# Autodesk Inventor assembly: SimulationWheelAssembly
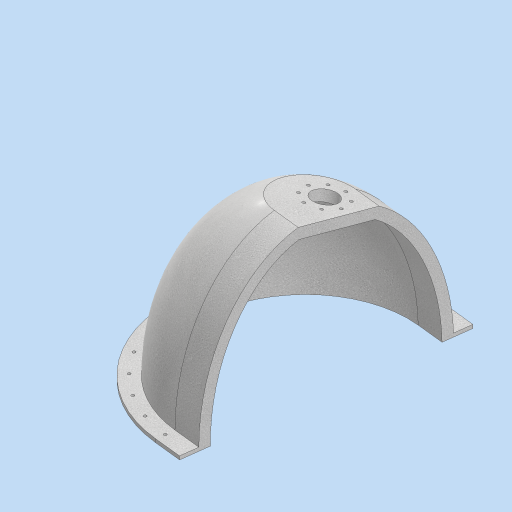
[picture p0: Inventor's stored thumbnail of the model, 512x512]
Saved by Autodesk Inventor 2023 (Build 270158000, 158)
## iProperties
Created: 2026-03-22
Part Number: SimulationWheelAssembly
Document SubType Name: Assembly
Designer: Nathann
Mass: 20175 g
Surface Area: 18221.2 cm^2
Volume: 20175 cm^3
Density: 1 g/cm^3
Author: Nathann
## Documents named in this file (8)
- C:\Users\Nathann\ClawdDrive\Objet3D\neodrive\neodrive-cad-ergonomic-v1\SimulationWheelAssembly.iam
- C:\Users\Nathann\ClawdDrive\Objet3D\neodrive\neodrive-cad-ergonomic-v1\eggshellCorePrintedLeft.ipt
- C:\Users\Nathann\ClawdDrive\Objet3D\neodrive\neodrive-cad-ergonomic-v1\SimulationWheelAssembly\AIP\FEA\fdktl59i8.fins
- C:\Users\Nathann\ClawdDrive\Objet3D\neodrive\neodrive-cad-ergonomic-v1\SimulationWheelAssembly\AIP\FEA\fdktl59i8.fsat
- C:\Users\Nathann\ClawdDrive\Objet3D\neodrive\neodrive-cad-ergonomic-v1\SimulationWheelAssembly\AIP\FEA\fdktl59j4.ftes
- C:\Users\Nathann\ClawdDrive\Objet3D\neodrive\neodrive-cad-ergonomic-v1\SimulationWheelAssembly\AIP\FEA\fdktl59j4.fwiz
- C:\Users\Nathann\ClawdDrive\Objet3D\neodrive\neodrive-cad-ergonomic-v1\SimulationWheelAssembly\AIP\FEA\fdktl59k0.fmsh
- C:\Users\Nathann\ClawdDrive\Objet3D\neodrive\neodrive-cad-ergonomic-v1\SimulationWheelAssembly\AIP\FEA\fdktl59k1.fres
## Components (1 placed, 1 different names)
1. eggshellCorePrintedLeft:1
## Named parameters: sa_0 = 300000, sa_1 = 0 mm, sa_2 = -700 mm, sa_3 = 0 mm, sa_4 = 300000
note: some values were not read from the file. Shown as the stored number, unit unknown: "sa_0", "sa_4".
